# Autodesk Inventor assembly: Y_rail_Assembly_Rev3
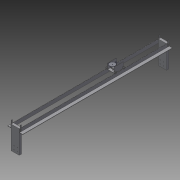
[picture p0: Inventor's stored thumbnail of the model, 180x180]
Saved by Autodesk Inventor 2015 (Build 190159000, 159)
## iProperties
Created: 2017-01-11
Part Number: Y_rail_Assembly_Rev3
Document SubType Name: Assembly
Designer: Guy
Author: Guy
## Documents named in this file (8)
- C:\Users\Guy\Documents\Fourth Year\Capstone\git\Capstone-Project\doc\CAD\LowLevel_Rev3\Y_rail_Assembly_Rev3.iam
- C:\Users\Guy\Documents\Fourth Year\Capstone\git\Capstone-Project\doc\CAD\LowLevel_Rev3\Y_Rail-SquareBar-Rev3.ipt
- C:\Users\Guy\Documents\Fourth Year\Capstone\git\Capstone-Project\doc\CAD\LowLevel_Rev3\Arm-SquareBar-Rev3.ipt
- C:\Users\Guy\Documents\Fourth Year\Capstone\git\Capstone-Project\doc\CAD\LowLevel_Rev3\XY_Wheel-SquareBar-Rev3.ipt
- C:\Users\Guy\Documents\Fourth Year\Capstone\git\Capstone-Project\doc\CAD\LowLevel_Rev3\EE_Base-SquareBar-Rev3.ipt
- C:\Users\Guy\Documents\Fourth Year\Capstone\git\Capstone-Project\doc\CAD\LowLevel_Rev3\Y_rail_Assembly_Rev3\Design Accelerator\Spur Gears1.iam
- C:\Users\Guy\Documents\Fourth Year\Capstone\git\Capstone-Project\doc\CAD\LowLevel_Rev3\Stepper_Motor_Holder-SquareBar-Rev3.ipt
- C:\Users\Guy\Documents\Fourth Year\Capstone\git\Capstone-Project\doc\CAD\LowLevel_Rev3\Y_Rail_Limit_Rod-SquareBar-Rev3.ipt
## Components (15 placed, 7 different names)
1. Y_Rail-SquareBar-Rev3:1 — Mate:2, Mate:5, Mate:6, Tangent:1, Tangent:2, Mate:11, Mate:24, Mate:25, Mate:26, Mate:27, Mate:28, Mate:29
2. Y_Rail-SquareBar-Rev3:2 — Mate:1, Mate:4, Mate:7, Mate:8, Tangent:3, Tangent:4, Mate:12, Mate:21, Mate:22, Mate:23, Mate:30, Mate:31, Mate:32
3. Arm-SquareBar-Rev3:1 — Mate:1, Mate:2, Mate:5, Flush:1, Mate:7
4. Arm-SquareBar-Rev3:2 — Mate:4, Mate:6, Flush:1, Mate:8
5. XY_Wheel-SquareBar-Rev3:1 — Tangent:1, Mate:9, Flush:2
6. XY_Wheel-SquareBar-Rev3:2 — Tangent:4, Mate:9, Flush:4, Mate:15, Mate:16
7. XY_Wheel-SquareBar-Rev3:3 — Tangent:3, Mate:10, Mate:12, Flush:4, Mate:14
8. XY_Wheel-SquareBar-Rev3:4 — Tangent:2, Mate:10, Mate:11, Flush:2, Mate:13
9. Spur Gears:1 [sub-assembly] — Mate:17
10. EE_Base-SquareBar-Rev3:1 — Mate:13, Mate:14, Mate:15, Mate:16, Mate:17, Mate:18, Mate:19, Mate:20
11. Stepper_Motor_Holder-SquareBar-Rev3:1 — Mate:18, Mate:19, Mate:20
12. Y_Rail_Limit_Rod-SquareBar-Rev3:2 — Mate:24, Mate:25, Mate:26
13. Y_Rail_Limit_Rod-SquareBar-Rev3:3 — Mate:21, Mate:22, Mate:23
14. Y_Rail_Limit_Rod-SquareBar-Rev3:4 — Mate:27, Mate:28, Mate:29
15. Y_Rail_Limit_Rod-SquareBar-Rev3:5 — Mate:30, Mate:31, Mate:32
## Relationships (38: Mate 31, Tangent 4, Flush 3)
- Mate:1: Y_Rail-SquareBar-Rev3:2 ↔ Arm-SquareBar-Rev3:1
- Mate:2: Y_Rail-SquareBar-Rev3:1 ↔ Arm-SquareBar-Rev3:1
- Mate:4: Y_Rail-SquareBar-Rev3:2 ↔ Arm-SquareBar-Rev3:2
- Mate:5: Y_Rail-SquareBar-Rev3:1 ↔ Arm-SquareBar-Rev3:1
- Mate:6: Y_Rail-SquareBar-Rev3:1 ↔ Arm-SquareBar-Rev3:2
- Flush:1: Arm-SquareBar-Rev3:1 ↔ Arm-SquareBar-Rev3:2
- Mate:7: Y_Rail-SquareBar-Rev3:2 ↔ Arm-SquareBar-Rev3:1
- Mate:8: Y_Rail-SquareBar-Rev3:2 ↔ Arm-SquareBar-Rev3:2
- Tangent:1: Y_Rail-SquareBar-Rev3:1 ↔ XY_Wheel-SquareBar-Rev3:1
- Tangent:2: Y_Rail-SquareBar-Rev3:1 ↔ XY_Wheel-SquareBar-Rev3:4
- Tangent:3: Y_Rail-SquareBar-Rev3:2 ↔ XY_Wheel-SquareBar-Rev3:3
- Tangent:4: Y_Rail-SquareBar-Rev3:2 ↔ XY_Wheel-SquareBar-Rev3:2
- Mate:9: XY_Wheel-SquareBar-Rev3:1 ↔ XY_Wheel-SquareBar-Rev3:2
- Mate:10: XY_Wheel-SquareBar-Rev3:3 ↔ XY_Wheel-SquareBar-Rev3:4
- Mate:11 (1.75 mm): Y_Rail-SquareBar-Rev3:1 ↔ XY_Wheel-SquareBar-Rev3:4
- Flush:2: XY_Wheel-SquareBar-Rev3:1 ↔ XY_Wheel-SquareBar-Rev3:4
- Mate:12 (1.75 mm): Y_Rail-SquareBar-Rev3:2 ↔ XY_Wheel-SquareBar-Rev3:3
- Flush:4: XY_Wheel-SquareBar-Rev3:2 ↔ XY_Wheel-SquareBar-Rev3:3
- Mate:13: XY_Wheel-SquareBar-Rev3:4 ↔ EE_Base-SquareBar-Rev3:1
- Mate:14: XY_Wheel-SquareBar-Rev3:3 ↔ EE_Base-SquareBar-Rev3:1
- Mate:15: XY_Wheel-SquareBar-Rev3:2 ↔ EE_Base-SquareBar-Rev3:1
- Mate:16 (2.25 mm): XY_Wheel-SquareBar-Rev3:2 ↔ EE_Base-SquareBar-Rev3:1
- Mate:17: Spur Gears:1 ↔ EE_Base-SquareBar-Rev3:1
- Mate:18: EE_Base-SquareBar-Rev3:1 ↔ Stepper_Motor_Holder-SquareBar-Rev3:1
- Mate:19: EE_Base-SquareBar-Rev3:1 ↔ Stepper_Motor_Holder-SquareBar-Rev3:1
- Mate:20: EE_Base-SquareBar-Rev3:1 ↔ Stepper_Motor_Holder-SquareBar-Rev3:1
- Mate:21: Y_Rail-SquareBar-Rev3:2 ↔ Y_Rail_Limit_Rod-SquareBar-Rev3:3
- Mate:22: Y_Rail-SquareBar-Rev3:2 ↔ Y_Rail_Limit_Rod-SquareBar-Rev3:3
- Mate:23: Y_Rail-SquareBar-Rev3:2 ↔ Y_Rail_Limit_Rod-SquareBar-Rev3:3
- Mate:24: Y_Rail-SquareBar-Rev3:1 ↔ Y_Rail_Limit_Rod-SquareBar-Rev3:2
- Mate:25: Y_Rail-SquareBar-Rev3:1 ↔ Y_Rail_Limit_Rod-SquareBar-Rev3:2
- Mate:26: Y_Rail-SquareBar-Rev3:1 ↔ Y_Rail_Limit_Rod-SquareBar-Rev3:2
- Mate:27: Y_Rail-SquareBar-Rev3:1 ↔ Y_Rail_Limit_Rod-SquareBar-Rev3:4
- Mate:28: Y_Rail-SquareBar-Rev3:1 ↔ Y_Rail_Limit_Rod-SquareBar-Rev3:4
- Mate:29: Y_Rail-SquareBar-Rev3:1 ↔ Y_Rail_Limit_Rod-SquareBar-Rev3:4
- Mate:30: Y_Rail-SquareBar-Rev3:2 ↔ Y_Rail_Limit_Rod-SquareBar-Rev3:5
- Mate:31: Y_Rail-SquareBar-Rev3:2 ↔ Y_Rail_Limit_Rod-SquareBar-Rev3:5
- Mate:32: Y_Rail-SquareBar-Rev3:2 ↔ Y_Rail_Limit_Rod-SquareBar-Rev3:5
